# Autodesk Inventor assembly: Assembly Spider Crab
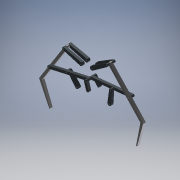
[picture p0: Inventor's stored thumbnail of the model, 180x180]
Saved by Autodesk Inventor 2019 (Build 230136000, 136)
## iProperties
Created: 2019-08-25
Part Number: Assembly Spider Crab
Document SubType Name: Assembly
Designer: DIBYOJYOTI
Author: DIBYOJYOTI
## Documents named in this file (9)
- D:\Autocad\Assembly Spider Crab.iam
- D:\Autocad\Crank.ipt
- D:\Autocad\Leg Spider Crab.ipt
- D:\Autocad\Lower Rocker Arm Spider Crab.ipt
- D:\Autocad\Rocker arm Leg Spider Crab.ipt
- D:\Autocad\Upper Rocker Arm Spider Crab.ipt
- D:\Autocad\Joint Pin Spider Crab.ipt
- D:\Autocad\Short Joint Pin Spider Crab.ipt
- D:\Autocad\Long Joint Pin Spider Crab.ipt
## Components (19 placed, 8 different names)
1. Leg Spider Crab:1 — Insert:7, Insert:15
2. Lower Rocker Arm Spider Crab:1 — Insert:12
3. Rocker arm Leg Spider Crab:1 — Insert:13, Insert:14, Insert:17
4. Crank:1 — Insert:16
5. Joint Pin Spider Crab:1 — Insert:7, Insert:8, Insert:9
6. Upper Rocker Arm Spider Crab:2 — Insert:8
7. Upper Rocker Arm Spider Crab:3 — Insert:9
8. Short Joint Pin Spider Crab:2 — Insert:12, Insert:13
9. Short Joint Pin Spider Crab:3 — Insert:14, Insert:15
10. Long Joint Pin Spider Crab:1 — Insert:16, Insert:17, Insert:25, Insert:26
11. Leg Spider Crab:2
12. Lower Rocker Arm Spider Crab:2
13. Rocker arm Leg Spider Crab:2 — Insert:25
14. Upper Rocker Arm Spider Crab:4
15. Joint Pin Spider Crab:2
16. Upper Rocker Arm Spider Crab:5
17. Short Joint Pin Spider Crab:4
18. Short Joint Pin Spider Crab:5
19. Crank:2 — Insert:26
## Relationships (18: Insert 18)
- Insert:7 (-11 mm): Leg Spider Crab:1 ↔ Joint Pin Spider Crab:1
- Insert:8: Joint Pin Spider Crab:1 ↔ Upper Rocker Arm Spider Crab:2
- Insert:9: Joint Pin Spider Crab:1 ↔ Upper Rocker Arm Spider Crab:3
- Insert:12: Lower Rocker Arm Spider Crab:1 ↔ Short Joint Pin Spider Crab:2
- Insert:13: Rocker arm Leg Spider Crab:1 ↔ Short Joint Pin Spider Crab:2
- Insert:14: Rocker arm Leg Spider Crab:1 ↔ Short Joint Pin Spider Crab:3
- Insert:15: Leg Spider Crab:1 ↔ Short Joint Pin Spider Crab:3
- Insert:16: Crank:1 ↔ Long Joint Pin Spider Crab:1
- Insert:17 (-22 mm): Rocker arm Leg Spider Crab:1 ↔ Long Joint Pin Spider Crab:1
- [Insert] (-11 mm): Leg Spider Crab:2 ↔ Joint Pin Spider Crab:2
- [Insert]: Upper Rocker Arm Spider Crab:4 ↔ Joint Pin Spider Crab:2
- [Insert]: Joint Pin Spider Crab:2 ↔ Upper Rocker Arm Spider Crab:5
- [Insert]: Lower Rocker Arm Spider Crab:2 ↔ Short Joint Pin Spider Crab:4
- [Insert]: Rocker arm Leg Spider Crab:2 ↔ Short Joint Pin Spider Crab:4
- [Insert]: Rocker arm Leg Spider Crab:2 ↔ Short Joint Pin Spider Crab:5
- [Insert]: Leg Spider Crab:2 ↔ Short Joint Pin Spider Crab:5
- Insert:25 (11 mm): Long Joint Pin Spider Crab:1 ↔ Rocker arm Leg Spider Crab:2
- Insert:26: Long Joint Pin Spider Crab:1 ↔ Crank:2
## Named parameters: d36_d32 = 0 mm, d37_d33 = 0 mm, d38_d27 = 0 mm, d39_d28 = 0 mm, d40_d16 = -11 mm, d41_d17 = 0 mm, d42_d19 = 0 mm
